(part 1 of 2)
# Autodesk Inventor assembly: testframe
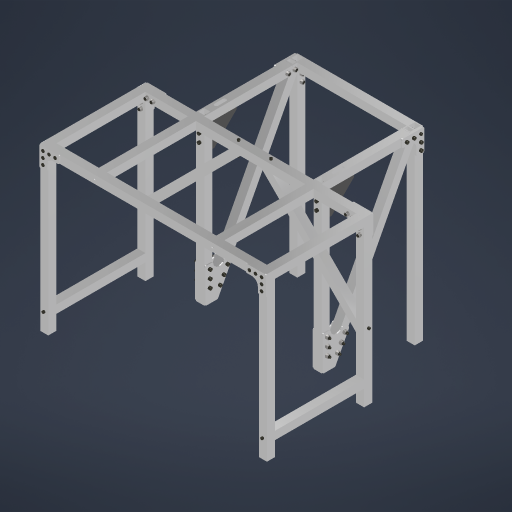
[picture p0: Inventor's stored thumbnail of the model, 512x512]
Saved by Autodesk Inventor 2024.2 (Build 282272000, 272)
## iProperties
Created: 2024-07-23
Part Number: testframe
Document SubType Name: Assembly
Designer: bryan
Mass: 9469.34 g
Surface Area: 20671.9 cm^2
Volume: 3372.68 cm^3
Density: 2.80766 g/cm^3
Author: bryan
## Documents named in this file (33)
- C:\Users\bobsb\OneDrive\Documents\GitHub\1622-2024-Summer-CAD-A-Thon\Structure\STRU_000_StructureAssembly.iam
- C:\Users\bobsb\OneDrive\Documents\GitHub\1622-2024-Summer-CAD-A-Thon\Structure\STRU_001_BilletBlock.ipt
- C:\Users\bobsb\OneDrive\Documents\GitHub\1622-2024-Summer-CAD-A-Thon\Structure\STRU_002_BilletPole_20.56in_Angled.ipt
- C:\Users\bobsb\OneDrive\Documents\GitHub\1622-2024-Summer-CAD-A-Thon\Structure\STRU_003_BilletPole_28in_Angled.ipt
- C:\Users\bobsb\OneDrive\Documents\GitHub\1622-2024-Summer-CAD-A-Thon\Structure\STRU_004_DoubleBillet_90_2.25in.ipt
- C:\Users\bobsb\OneDrive\Documents\GitHub\1622-2024-Summer-CAD-A-Thon\Structure\STRU_007_BilletPole_11in.ipt
- C:\Users\bobsb\OneDrive\Documents\GitHub\1622-2024-Summer-CAD-A-Thon\Structure\STRU_003_BilletPole_28in_Angled_Unique.ipt
- C:\Users\bobsb\OneDrive\Documents\GitHub\1622-2024-Summer-CAD-A-Thon\COTS Library\Fasteners\Bolts\Socket-Head\10-32\COTS_90044A120_Black-Oxide Alloy Steel Socket Head Screw.ipt
- C:\Users\bobsb\OneDrive\Documents\GitHub\1622-2024-Summer-CAD-A-Thon\COTS Library\Fasteners\Bolts\Socket-Head\0.25-20\COTS_90044A123_Black-Oxide Alloy Steel Socket Head Screw.ipt
- C:\Users\bobsb\OneDrive\Documents\GitHub\1622-2024-Summer-CAD-A-Thon\COTS Library\Fasteners\Nuts\COTS_95615A120_Medium-Strength Steel Nylon-Insert Locknut.ipt
- C:\Users\bobsb\OneDrive\Documents\GitHub\1622-2024-Summer-CAD-A-Thon\Structure\STRU_009_FrameBracket_90.ipt
- C:\Users\bobsb\OneDrive\Documents\GitHub\1622-2024-Summer-CAD-A-Thon\Structure\STRU_006_BilletPole_SwerveOffset.ipt
- C:\Users\bobsb\OneDrive\Documents\GitHub\1622-2024-Summer-CAD-A-Thon\Structure\STRU_010_BilletCrossbar_Angled.ipt
- C:\Users\bobsb\OneDrive\Documents\GitHub\1622-2024-Summer-CAD-A-Thon\Structure\STRU_011_BilletWedge.ipt
- C:\Users\bobsb\OneDrive\Documents\GitHub\1622-2024-Summer-CAD-A-Thon\COTS Library\Fasteners\Bolts\Socket-Head\10-32\COTS_90044A119_Black-Oxide Alloy Steel Socket Head Screw.ipt
- C:\Users\bobsb\OneDrive\Documents\GitHub\1622-2024-Summer-CAD-A-Thon\Structure\STRU_012_BilletPoleMiddle.ipt
- C:\Users\bobsb\OneDrive\Documents\GitHub\1622-2024-Summer-CAD-A-Thon\Structure\STRU_013_BilletCrossbar2_Angled.ipt
- C:\Users\bobsb\OneDrive\Documents\GitHub\1622-2024-Summer-CAD-A-Thon\Structure\STRU_012_BilletPoleMiddle_Unique.ipt
- C:\Users\bobsb\OneDrive\Documents\GitHub\1622-2024-Summer-CAD-A-Thon\Structure\STRU_014_BilletPole_9in_Angled.ipt
- C:\Users\bobsb\OneDrive\Documents\GitHub\1622-2024-Summer-CAD-A-Thon\Structure\STRU_015_BilletPole_9in.ipt
- C:\Users\bobsb\OneDrive\Documents\GitHub\1622-2024-Summer-CAD-A-Thon\Structure\STRU_016_FrameBracket2_90.ipt
- C:\Users\bobsb\OneDrive\Documents\GitHub\1622-2024-Summer-CAD-A-Thon\Structure\STRU_017_AngleBracket_90_Plastic.ipt
- C:\Users\bobsb\OneDrive\Documents\GitHub\1622-2024-Summer-CAD-A-Thon\Structure\STRU_018_AngleBracket_62.ipt
- C:\Users\bobsb\OneDrive\Documents\GitHub\1622-2024-Summer-CAD-A-Thon\COTS Library\Fasteners\Bolts\Socket-Head\0.25-20\COTS_91251A539_Black-Oxide Alloy Steel Socket Head Screw (1).ipt
- C:\Users\bobsb\OneDrive\Documents\GitHub\1622-2024-Summer-CAD-A-Thon\COTS Library\Fasteners\Bolts\Socket-Head\0.25-20\COTS_90044A124_Black-Oxide Alloy Steel Socket Head Screw.ipt
- C:\Users\bobsb\OneDrive\Documents\GitHub\1622-2024-Summer-CAD-A-Thon\COTS Library\Fasteners\Nuts\COTS_95462A029_Medium-Strength Steel Hex Nut (2).ipt
- C:\Users\bobsb\OneDrive\Documents\GitHub\1622-2024-Summer-CAD-A-Thon\Structure\STRU_019_RubberWasher.ipt
- C:\Users\bobsb\OneDrive\Documents\GitHub\1622-2024-Summer-CAD-A-Thon\Structure\STRU_023_Kenji_11in.ipt
- C:\Users\bobsb\OneDrive\Documents\GitHub\1622-2024-Summer-CAD-A-Thon\Structure\STRU_024_BilletBlock2.ipt
- C:\Users\bobsb\OneDrive\Documents\GitHub\1622-2024-Summer-CAD-A-Thon\COTS Library\Fasteners\Bolts\Socket-Head\0.25-20\COTS_90357A018_Ultra-Low-Profile Socket Head Screw.ipt
- C:\Users\bobsb\OneDrive\Documents\GitHub\1622-2024-Summer-CAD-A-Thon\COTS Library\Fasteners\Bolts\Socket-Head\0.25-20\COTS_90357A021_Ultra-Low-Profile Socket Head Screw.ipt
- C:\Users\bobsb\OneDrive\Documents\GitHub\1622-2024-Summer-CAD-A-Thon\COTS Library\Fasteners\Bolts\Socket-Head\10-32\COTS_91251A352_Black-Oxide Alloy Steel Socket Head.ipt
- C:\Users\bobsb\OneDrive\Documents\GitHub\1622-2024-Summer-CAD-A-Thon\Structure\STRU_000_StructureAssembly\AIP\FEA\err5tqxb5.fres
## Components (177 placed, 31 different names)
1. STRU_001_BilletBlock:2 — Mate:16, Mate:17, Flush:2
2. STRU_002_BilletPole_20.56in_Angled:1 — Mate:1, Mate:4, Mate:5, Mate:41, Mate:53, Mate:54, Flush:10, Mate:91, Mate:92, Mate:127, Mate:147, Mate:148, Mate:209, Mate:211, Mate:212, Mate:213, Mate:411, Mate:470, Mate:471, Flush:63, Mate:527, Mate:528
3. STRU_004_DoubleBillet_90_2.25in:1 — Mate:1, Mate:4, Mate:5, Mate:34, Mate:56, Mate:58, Mate:125, Mate:126
4. STRU_002_BilletPole_20.56in_Angled:2 — Mate:13, Mate:14, Mate:15, Mate:16, Mate:17, Flush:2, Mate:40, Mate:85, Mate:86, Mate:123, Mate:124, Mate:145, Mate:146, Mate:200, Mate:201, Mate:218, Mate:219, Mate:415, Mate:477, Mate:478, Mate:483, Mate:531, Mate:532
5. STRU_004_DoubleBillet_90_2.25in:2 — Mate:13, Mate:14, Mate:15, Mate:36, Mate:57, Mate:100, Mate:121, Mate:122
6. STRU_001_BilletBlock:3 — Mate:185, Mate:186, Flush:26
7. STRU_001_BilletBlock:4 — Mate:180, Mate:181, Flush:25
8. STRU_003_BilletPole_28in_Angled:2 — Mate:47, Flush:8, Flush:9, Mate:55, Mate:118, Mate:130, Mate:153, Mate:154, Mate:155, Mate:156, Mate:173, Flush:24, Mate:176, Mate:178, Mate:182, Mate:484, Mate:485, Mate:486, Mate:490, Flush:68, Mate:491, Mate:492, Mate:493
9. STRU_004_DoubleBillet_90_2.25in:3 — Mate:128, Mate:129, Mate:184
10. STRU_004_DoubleBillet_90_2.25in:4 — Mate:119, Mate:120, Mate:179
11. STRU_001_BilletBlock:5 — Mate:34, Mate:41, Mate:50, Mate:51, Flush:65
12. STRU_001_BilletBlock:8 — Mate:36, Mate:40, Mate:42, Mate:43
13. STRU_007_BilletPole_11in:1 — Flush:9, Mate:50, Mate:51, Mate:55, Mate:59
14. STRU_007_BilletPole_11in:2 — Mate:42, Mate:43, Mate:47, Flush:8, Mate:124
15. STRU_001_BilletBlock:9 — Mate:53, Mate:54, Flush:10
16. STRU_003_BilletPole_28in_Angled_Unique:1 — Mate:56, Mate:57, Mate:58, Mate:59, Mate:83, Mate:84, Mate:93, Mate:94, Mate:98, Mate:149, Mate:150, Mate:151, Mate:152, Mate:159, Mate:160, Mate:164, Mate:165, Flush:27, Mate:203, Mate:205, Mate:206, Mate:208, Mate:214, Mate:215, Mate:216, Mate:217, Flush:28, Mate:221, Flush:29, Mate:223, Mate:261, Mate:262, Mate:408, Mate:412, Flush:68
17. COTS_90044A123_Black-Oxide Alloy Steel Socket Head Screw:6 — Mate:84, Mate:108, Flush:12
18. COTS_90044A123_Black-Oxide Alloy Steel Socket Head Screw:7 — Mate:85, Mate:106, Mate:134, Flush:12, Flush:13, Flush:14
19. COTS_90044A123_Black-Oxide Alloy Steel Socket Head Screw:8 — Mate:83, Mate:107, Flush:13
20. COTS_90044A123_Black-Oxide Alloy Steel Socket Head Screw:9 — Mate:86, Mate:105, Flush:14
21. COTS_90044A123_Black-Oxide Alloy Steel Socket Head Screw:14 — Mate:93, Mate:115, Flush:16
22. COTS_90044A123_Black-Oxide Alloy Steel Socket Head Screw:15 — Mate:92, Mate:114, Flush:17
23. COTS_90044A123_Black-Oxide Alloy Steel Socket Head Screw:16 — Mate:91, Mate:113, Mate:136, Flush:15, Flush:17
24. COTS_90044A123_Black-Oxide Alloy Steel Socket Head Screw:17 — Mate:94, Mate:116, Flush:15, Flush:16
25. COTS_90044A120_Black-Oxide Alloy Steel Socket Head Screw:6 — Mate:100, Mate:135
26. COTS_90044A120_Black-Oxide Alloy Steel Socket Head Screw:7 — Mate:98, Mate:137
27. COTS_95615A120_Medium-Strength Steel Nylon-Insert Locknut:1 — Mate:154, Mate:522
28. COTS_95615A120_Medium-Strength Steel Nylon-Insert Locknut:2 — Mate:153, Mate:521
29. COTS_95615A120_Medium-Strength Steel Nylon-Insert Locknut:3 — Mate:194, Mate:519
30. COTS_95615A120_Medium-Strength Steel Nylon-Insert Locknut:4 — Mate:195, Mate:520
31. COTS_95615A120_Medium-Strength Steel Nylon-Insert Locknut:5 — Mate:107, Mate:152
32. COTS_95615A120_Medium-Strength Steel Nylon-Insert Locknut:6 — Mate:108, Mate:151
33. COTS_95615A120_Medium-Strength Steel Nylon-Insert Locknut:7 — Mate:105, Mate:145
34. COTS_95615A120_Medium-Strength Steel Nylon-Insert Locknut:8 — Mate:106, Mate:146
35. COTS_95615A120_Medium-Strength Steel Nylon-Insert Locknut:9 — Mate:155, Mate:514
36. COTS_95615A120_Medium-Strength Steel Nylon-Insert Locknut:10 — Mate:156, Mate:515
37. COTS_95615A120_Medium-Strength Steel Nylon-Insert Locknut:11 — Mate:189, Mate:513
38. COTS_95615A120_Medium-Strength Steel Nylon-Insert Locknut:12 — Mate:190, Mate:512
39. COTS_95615A120_Medium-Strength Steel Nylon-Insert Locknut:13 — Mate:114, Mate:147
40. COTS_95615A120_Medium-Strength Steel Nylon-Insert Locknut:14 — Mate:113, Mate:148
41. COTS_95615A120_Medium-Strength Steel Nylon-Insert Locknut:15 — Mate:115, Mate:149
42. COTS_95615A120_Medium-Strength Steel Nylon-Insert Locknut:16 — Mate:116, Mate:150
43. STRU_009_FrameBracket_90:1 — Mate:118, Mate:119, Mate:120, Mate:177, Mate:497, Mate:498, Mate:499, Mate:500, Mate:501, Mate:502, Mate:503, Mate:516, Mate:517, Mate:518
44. STRU_009_FrameBracket_90:2 — Mate:125, Mate:126, Mate:127, Mate:136, Mate:137
45. STRU_009_FrameBracket_90:3 — Mate:121, Mate:122, Mate:123, Mate:134, Mate:135
46. STRU_009_FrameBracket_90:4 — Mate:128, Mate:129, Mate:130, Mate:183, Mate:504, Mate:505, Mate:506, Mate:507, Mate:508, Mate:509, Mate:510, Mate:511, Mate:523, Mate:524
47. STRU_001_BilletBlock:11 — Mate:159, Mate:165, Mate:171
48. STRU_001_BilletBlock:12 — Mate:160, Mate:164, Mate:174, Flush:66
49. STRU_007_BilletPole_11in:3 — Mate:171, Mate:173, Flush:27
50. STRU_007_BilletPole_11in:4 — Mate:174, Flush:24, Mate:176
51. STRU_006_BilletPole_SwerveOffset:1 — Mate:177, Mate:178, Mate:179, Mate:180, Mate:181, Flush:25, Mate:194, Mate:195, Flush:64, Mate:487, Mate:489, Mate:494, Mate:529, Mate:530
52. STRU_006_BilletPole_SwerveOffset:2 — Mate:182, Mate:183, Mate:184, Mate:185, Mate:186, Flush:26, Mate:189, Mate:190, Mate:475, Mate:488, Mate:495, Mate:525, Mate:526
53. STRU_011_BilletWedge:1 — Mate:200, Mate:201, Mate:414
54. STRU_011_BilletWedge:3 — Mate:203, Mate:205, Mate:413
55. STRU_011_BilletWedge:4 — Mate:206, Mate:208, Mate:409
56. STRU_011_BilletWedge:5 — Mate:209, Mate:211, Mate:410
57. COTS_90044A119_Black-Oxide Alloy Steel Socket Head Screw:1 — Mate:212, Mate:213
58. COTS_90044A119_Black-Oxide Alloy Steel Socket Head Screw:2 — Mate:214, Mate:215
59. COTS_90044A119_Black-Oxide Alloy Steel Socket Head Screw:3 — Mate:216, Mate:217
60. COTS_90044A119_Black-Oxide Alloy Steel Socket Head Screw:4 — Mate:218, Mate:219
61. STRU_012_BilletPoleMiddle:6 — Flush:28, Mate:221, Mate:228, Mate:229, Flush:30, Flush:43, Mate:251, Mate:255, Flush:49, Mate:261, Mate:263, Mate:318, Mate:324, Mate:331, Mate:389, Mate:390, Mate:418, Mate:419
62. STRU_012_BilletPoleMiddle:5 — Flush:29, Mate:223, Mate:230, Mate:231, Flush:31, Flush:39, Mate:233, Mate:234, Mate:249, Mate:253, Flush:48, Mate:262, Mate:264, Mate:319, Mate:321, Mate:328, Mate:391, Mate:392, Mate:416, Mate:417
63. STRU_001_BilletBlock:14 — Mate:228, Mate:229, Flush:30
64. STRU_001_BilletBlock:15 — Mate:230, Mate:231, Flush:31
65. STRU_013_BilletCrossbar2_Angled:1 — Flush:39, Mate:233, Mate:234, Mate:252, Mate:273, Flush:56, Flush:57, Mate:287, Mate:322, Mate:323, Mate:327, Mate:329
66. STRU_013_BilletCrossbar2_Angled:3 — Flush:43, Mate:254, Mate:274, Flush:58, Mate:308, Mate:325, Mate:326, Mate:330, Mate:332
67. STRU_001_BilletBlock:16 — Mate:267, Mate:268, Flush:54
68. STRU_001_BilletBlock:17 — Mate:269, Mate:270, Flush:55
69. COTS_90044A120_Black-Oxide Alloy Steel Socket Head Screw:11 — Mate:249, Mate:264
70. COTS_90044A120_Black-Oxide Alloy Steel Socket Head Screw:12 — Mate:251, Mate:263
71. STRU_014_BilletPole_9in_Angled:1 — Mate:254, Mate:255, Flush:49, Mate:311, Mate:317, Mate:333, Mate:334, Mate:335, Mate:336
72. STRU_014_BilletPole_9in_Angled:2 — Mate:252, Mate:253, Flush:48, Mate:291, Mate:320, Mate:337, Mate:338, Mate:339, Mate:340
73. STRU_015_BilletPole_9in:1 — Mate:257, Mate:258, Mate:259, Mate:260, Flush:52, Flush:53, Flush:57
74. STRU_001_BilletBlock:18 — Mate:259, Mate:260, Flush:52, Mate:266, Mate:271, Mate:275
75. STRU_001_BilletBlock:19 — Mate:257, Mate:258, Flush:53, Mate:265, Mate:272, Mate:276
76. STRU_012_BilletPoleMiddle_Unique:1 — Mate:265, Mate:267, Mate:268, Flush:54, Mate:272, Mate:274, Flush:58, Mate:277, Mate:278, Mate:279, Mate:304, Mate:316
77. STRU_012_BilletPoleMiddle_Unique:2 — Mate:266, Mate:269, Mate:270, Flush:55, Mate:271, Mate:273, Flush:56, Mate:281, Mate:282, Mate:283, Mate:295, Mate:299
78. COTS_90044A120_Black-Oxide Alloy Steel Socket Head Screw:13 — Mate:275, Mate:284
79. COTS_90044A120_Black-Oxide Alloy Steel Socket Head Screw:14 — Mate:276, Mate:280
80. STRU_016_FrameBracket2_90:1 — Mate:277, Mate:278, Mate:279, Mate:280, Mate:302, Mate:303, Mate:306, Mate:307, Mate:310, Mate:312, Mate:314, Mate:315
81. STRU_016_FrameBracket2_90:2 — Mate:281, Mate:282, Mate:283, Mate:284, Mate:286, Mate:288, Mate:290, Mate:292, Mate:294, Mate:296, Mate:298, Mate:300
82. COTS_90044A123_Black-Oxide Alloy Steel Socket Head Screw:18 — Mate:286, Mate:288
83. COTS_95615A120_Medium-Strength Steel Nylon-Insert Locknut:17 — Mate:287
84. COTS_90044A123_Black-Oxide Alloy Steel Socket Head Screw:19 — Mate:290, Mate:292
85. COTS_95615A120_Medium-Strength Steel Nylon-Insert Locknut:18 — Mate:291
86. COTS_90044A123_Black-Oxide Alloy Steel Socket Head Screw:20 — Mate:294, Mate:296
87. COTS_95615A120_Medium-Strength Steel Nylon-Insert Locknut:19 — Mate:295
88. COTS_90044A123_Black-Oxide Alloy Steel Socket Head Screw:21 — Mate:298, Mate:300
89. COTS_95615A120_Medium-Strength Steel Nylon-Insert Locknut:20 — Mate:299
90. COTS_90044A123_Black-Oxide Alloy Steel Socket Head Screw:22 — Mate:302, Mate:303
91. COTS_95615A120_Medium-Strength Steel Nylon-Insert Locknut:21 — Mate:304
92. COTS_90044A123_Black-Oxide Alloy Steel Socket Head Screw:23 — Mate:306, Mate:307
93. COTS_95615A120_Medium-Strength Steel Nylon-Insert Locknut:22 — Mate:308
94. COTS_90044A123_Black-Oxide Alloy Steel Socket Head Screw:24 — Mate:310, Mate:312
95. COTS_95615A120_Medium-Strength Steel Nylon-Insert Locknut:23 — Mate:311
96. COTS_90044A123_Black-Oxide Alloy Steel Socket Head Screw:25 — Mate:314, Mate:315
97. COTS_95615A120_Medium-Strength Steel Nylon-Insert Locknut:24 — Mate:316
98. STRU_017_AngleBracket_90_Plastic:1 — Mate:317, Mate:318, Mate:453, Mate:454, Mate:458, Mate:462, Mate:463, Mate:467
99. STRU_017_AngleBracket_90_Plastic:2 — Mate:319, Mate:320, Mate:434, Mate:435, Mate:440, Mate:444, Mate:445, Mate:449
100. STRU_018_AngleBracket_62:1 — Mate:327, Mate:328, Mate:329, Mate:393, Mate:394, Mate:395, Mate:396, Mate:397, Mate:398, Mate:399, Mate:400, Mate:401, Mate:402, Mate:403, Mate:404
101. STRU_018_AngleBracket_62:2 — Mate:330, Mate:331, Mate:332, Mate:359, Mate:360, Mate:361, Mate:362, Mate:363, Mate:364, Mate:383, Mate:384, Mate:385, Mate:386, Mate:387, Mate:388
102. STRU_018_AngleBracket_62:3 — Mate:321, Mate:322, Mate:323, Mate:426, Mate:427, Mate:428, Mate:429, Mate:430, Mate:431
103. STRU_018_AngleBracket_62:4 — Mate:324, Mate:325, Mate:326, Mate:377, Mate:378, Mate:379, Mate:380, Mate:381, Mate:382
104. COTS_91251A539_Black-Oxide Alloy Steel Socket Head Screw (1):1 — Mate:337, Mate:340, Mate:439
105. COTS_91251A539_Black-Oxide Alloy Steel Socket Head Screw (1):2 — Mate:338, Mate:339, Mate:432, Mate:433
106. COTS_91251A539_Black-Oxide Alloy Steel Socket Head Screw (1):4 — Mate:333, Mate:334, Mate:457
107. COTS_91251A539_Black-Oxide Alloy Steel Socket Head Screw (1):5 — Mate:335, Mate:336, Mate:452
108. COTS_95615A120_Medium-Strength Steel Nylon-Insert Locknut:25 — Mate:373, Mate:385
109. COTS_95615A120_Medium-Strength Steel Nylon-Insert Locknut:26 — Mate:372, Mate:384
110. COTS_95615A120_Medium-Strength Steel Nylon-Insert Locknut:27 — Mate:371, Mate:383
111. COTS_95615A120_Medium-Strength Steel Nylon-Insert Locknut:28 — Mate:376, Mate:388
112. COTS_95615A120_Medium-Strength Steel Nylon-Insert Locknut:29 — Mate:375, Mate:387
113. COTS_95615A120_Medium-Strength Steel Nylon-Insert Locknut:30 — Mate:374, Mate:386
114. COTS_90044A123_Black-Oxide Alloy Steel Socket Head Screw:27 — Mate:390, Mate:419, Mate:461
115. COTS_90044A123_Black-Oxide Alloy Steel Socket Head Screw:28 — Mate:389, Mate:418, Mate:466
116. COTS_90044A123_Black-Oxide Alloy Steel Socket Head Screw:29 — Mate:392, Mate:417, Mate:448
117. COTS_90044A123_Black-Oxide Alloy Steel Socket Head Screw:30 — Mate:391, Mate:416, Mate:442, Mate:443
118. COTS_90044A124_Black-Oxide Alloy Steel Socket Head Screw:1 — Mate:359, Mate:371, Mate:382
119. COTS_90044A124_Black-Oxide Alloy Steel Socket Head Screw:2 — Mate:361, Mate:373, Mate:378
120. COTS_90044A124_Black-Oxide Alloy Steel Socket Head Screw:3 — Mate:360, Mate:372, Mate:381
121. COTS_90044A124_Black-Oxide Alloy Steel Socket Head Screw:4 — Mate:393, Mate:399, Mate:421
122. COTS_90044A124_Black-Oxide Alloy Steel Socket Head Screw:5 — Mate:394, Mate:401, Mate:422
123. COTS_90044A124_Black-Oxide Alloy Steel Socket Head Screw:6 — Mate:395, Mate:400, Mate:423
124. COTS_90044A124_Black-Oxide Alloy Steel Socket Head Screw:7 — Mate:362, Mate:374, Mate:379
125. COTS_90044A124_Black-Oxide Alloy Steel Socket Head Screw:8 — Mate:363, Mate:375, Mate:380
126. COTS_90044A124_Black-Oxide Alloy Steel Socket Head Screw:9 — Mate:364, Mate:376, Mate:377
127. COTS_90044A124_Black-Oxide Alloy Steel Socket Head Screw:10 — Mate:396, Mate:404, Mate:425
128. COTS_90044A124_Black-Oxide Alloy Steel Socket Head Screw:11 — Mate:397, Mate:403, Mate:424
129. COTS_90044A124_Black-Oxide Alloy Steel Socket Head Screw:12 — Mate:398, Mate:402, Mate:420
130. STRU_010_BilletCrossbar_Angled:2 — Mate:408, Mate:409, Mate:410, Mate:411
131. STRU_010_BilletCrossbar_Angled:3 — Mate:412, Mate:413, Mate:414, Mate:415
132. COTS_95615A120_Medium-Strength Steel Nylon-Insert Locknut:31 — Mate:423, Mate:430
133. COTS_95615A120_Medium-Strength Steel Nylon-Insert Locknut:32 — Mate:421, Mate:426
134. COTS_95615A120_Medium-Strength Steel Nylon-Insert Locknut:33 — Mate:425, Mate:429
135. COTS_95615A120_Medium-Strength Steel Nylon-Insert Locknut:34 — Mate:420, Mate:427
136. COTS_95615A120_Medium-Strength Steel Nylon-Insert Locknut:35 — Mate:422, Mate:431
137. COTS_95615A120_Medium-Strength Steel Nylon-Insert Locknut:36 — Mate:424, Mate:428
138. COTS_95462A029_Medium-Strength Steel Hex Nut (2):1 — Mate:432, Mate:436
139. STRU_019_RubberWasher:1 — Mate:433, Mate:434, Mate:435, Mate:436, Flush:59
140. COTS_95462A029_Medium-Strength Steel Hex Nut (2):2 — Mate:438, Mate:439
141. STRU_019_RubberWasher:2 — Mate:438, Flush:59, Mate:440
142. COTS_95462A029_Medium-Strength Steel Hex Nut (2):3 — Mate:442
143. STRU_019_RubberWasher:3 — Mate:443, Mate:444, Mate:445, Flush:60
144. COTS_95462A029_Medium-Strength Steel Hex Nut (2):4 — Mate:447, Mate:448
145. STRU_019_RubberWasher:4 — Mate:447, Mate:449, Flush:60
146. COTS_95462A029_Medium-Strength Steel Hex Nut (2):5 — Mate:452
147. STRU_019_RubberWasher:5 — Mate:453, Mate:454, Flush:61
148. COTS_95462A029_Medium-Strength Steel Hex Nut (2):6 — Mate:457
149. STRU_019_RubberWasher:6 — Mate:458, Flush:61
150. COTS_95462A029_Medium-Strength Steel Hex Nut (2):7 — Mate:461
151. STRU_019_RubberWasher:7 — Mate:462, Mate:463, Flush:62
152. COTS_95462A029_Medium-Strength Steel Hex Nut (2):8 — Mate:466
153. STRU_019_RubberWasher:8 — Mate:467, Flush:62
154. STRU_023_Kenji_11in:1 — Mate:472, Mate:473, Flush:63, Mate:475
155. STRU_023_Kenji_11in:2 — Flush:64, Mate:482, Mate:483, Mate:496
156. STRU_001_BilletBlock:22 — Mate:470, Mate:471, Mate:472, Mate:473
157. STRU_001_BilletBlock:23 — Mate:477, Mate:478, Mate:482
158. STRU_024_BilletBlock2:1 — Mate:484, Mate:490, Flush:65
159. STRU_024_BilletBlock2:2 — Mate:487, Flush:69, Mate:492
160. STRU_024_BilletBlock2:3 — Mate:488, Mate:495, Flush:70
161. STRU_024_BilletBlock2:4 — Mate:489, Mate:494, Flush:70, Mate:496
162. STRU_024_BilletBlock2:5 — Mate:486, Flush:67, Flush:69, Mate:491
163. STRU_024_BilletBlock2:6 — Mate:485, Flush:66, Flush:67, Mate:493
164. COTS_90357A018_Ultra-Low-Profile Socket Head Screw:1 — Mate:499, Mate:500, Mate:521
165. COTS_90357A021_Ultra-Low-Profile Socket Head Screw:1 — Mate:497, Mate:498
166. COTS_90357A018_Ultra-Low-Profile Socket Head Screw:2 — Mate:501, Mate:516, Mate:522
167. COTS_90357A018_Ultra-Low-Profile Socket Head Screw:3 — Mate:502, Mate:518, Mate:519
168. COTS_90357A018_Ultra-Low-Profile Socket Head Screw:4 — Mate:503, Mate:517, Mate:520
169. COTS_90357A018_Ultra-Low-Profile Socket Head Screw:5 — Mate:504, Mate:508, Mate:514
170. COTS_90357A018_Ultra-Low-Profile Socket Head Screw:6 — Mate:505, Mate:509, Mate:515
171. COTS_90357A018_Ultra-Low-Profile Socket Head Screw:7 — Mate:506, Mate:510, Mate:513
172. COTS_90357A018_Ultra-Low-Profile Socket Head Screw:8 — Mate:507, Mate:511, Mate:512
173. COTS_90357A021_Ultra-Low-Profile Socket Head Screw:2 — Mate:523, Mate:524
174. COTS_91251A352_Black-Oxide Alloy Steel Socket Head:1 — Mate:525, Mate:526
175. COTS_91251A352_Black-Oxide Alloy Steel Socket Head:2 — Mate:527, Mate:528
176. COTS_91251A352_Black-Oxide Alloy Steel Socket Head:3 — Mate:529, Mate:530
177. COTS_91251A352_Black-Oxide Alloy Steel Socket Head:4 — Mate:531, Mate:532
## Relationships (412: Mate 371, Flush 41)
- Mate:1: STRU_002_BilletPole_20.56in_Angled:1 ↔ STRU_004_DoubleBillet_90_2.25in:1
- Mate:4: STRU_002_BilletPole_20.56in_Angled:1 ↔ STRU_004_DoubleBillet_90_2.25in:1
- Mate:5: STRU_002_BilletPole_20.56in_Angled:1 ↔ STRU_004_DoubleBillet_90_2.25in:1
- Mate:13: STRU_002_BilletPole_20.56in_Angled:2 ↔ STRU_004_DoubleBillet_90_2.25in:2
- Mate:14: STRU_002_BilletPole_20.56in_Angled:2 ↔ STRU_004_DoubleBillet_90_2.25in:2
- Mate:15: STRU_002_BilletPole_20.56in_Angled:2 ↔ STRU_004_DoubleBillet_90_2.25in:2
- Mate:16: STRU_001_BilletBlock:2 ↔ STRU_002_BilletPole_20.56in_Angled:2
- Mate:17: STRU_001_BilletBlock:2 ↔ STRU_002_BilletPole_20.56in_Angled:2
- Flush:2: STRU_001_BilletBlock:2 ↔ STRU_002_BilletPole_20.56in_Angled:2
- [Mate]: STRU_003_BilletPole_28in_Angled:2 ↔ STRU_004_DoubleBillet_90_2.25in:3
- [Mate]: STRU_003_BilletPole_28in_Angled:2 ↔ STRU_004_DoubleBillet_90_2.25in:3
- [Mate]: STRU_003_BilletPole_28in_Angled:2 ↔ STRU_004_DoubleBillet_90_2.25in:3
- [Mate]: STRU_003_BilletPole_28in_Angled:2 ↔ STRU_004_DoubleBillet_90_2.25in:4
- [Mate]: STRU_003_BilletPole_28in_Angled:2 ↔ STRU_004_DoubleBillet_90_2.25in:4
- [Mate]: STRU_003_BilletPole_28in_Angled:2 ↔ STRU_004_DoubleBillet_90_2.25in:4
- Mate:34: STRU_004_DoubleBillet_90_2.25in:1 ↔ STRU_001_BilletBlock:5
- Mate:36: STRU_004_DoubleBillet_90_2.25in:2 ↔ STRU_001_BilletBlock:8
- Mate:40: STRU_002_BilletPole_20.56in_Angled:2 ↔ STRU_001_BilletBlock:8
- Mate:41: STRU_002_BilletPole_20.56in_Angled:1 ↔ STRU_001_BilletBlock:5
- Mate:42: STRU_001_BilletBlock:8 ↔ STRU_007_BilletPole_11in:2
- Mate:43: STRU_001_BilletBlock:8 ↔ STRU_007_BilletPole_11in:2
- Mate:47: STRU_003_BilletPole_28in_Angled:2 ↔ STRU_007_BilletPole_11in:2
- Flush:8: STRU_003_BilletPole_28in_Angled:2 ↔ STRU_007_BilletPole_11in:2
- Flush:9: STRU_003_BilletPole_28in_Angled:2 ↔ STRU_007_BilletPole_11in:1
- Mate:50: STRU_001_BilletBlock:5 ↔ STRU_007_BilletPole_11in:1
- Mate:51: STRU_001_BilletBlock:5 ↔ STRU_007_BilletPole_11in:1
- Mate:53: STRU_002_BilletPole_20.56in_Angled:1 ↔ STRU_001_BilletBlock:9
- Mate:54: STRU_002_BilletPole_20.56in_Angled:1 ↔ STRU_001_BilletBlock:9
- Flush:10: STRU_002_BilletPole_20.56in_Angled:1 ↔ STRU_001_BilletBlock:9
- Mate:55: STRU_003_BilletPole_28in_Angled:2 ↔ STRU_007_BilletPole_11in:1
- Mate:56: STRU_004_DoubleBillet_90_2.25in:1 ↔ STRU_003_BilletPole_28in_Angled_Unique:1
- Mate:57: STRU_004_DoubleBillet_90_2.25in:2 ↔ STRU_003_BilletPole_28in_Angled_Unique:1
- Mate:58: STRU_004_DoubleBillet_90_2.25in:1 ↔ STRU_003_BilletPole_28in_Angled_Unique:1
- Mate:59: STRU_007_BilletPole_11in:1 ↔ STRU_003_BilletPole_28in_Angled_Unique:1
- Mate:83: STRU_003_BilletPole_28in_Angled_Unique:1 ↔ COTS_90044A123_Black-Oxide Alloy Steel Socket Head Screw:8
- Mate:84: STRU_003_BilletPole_28in_Angled_Unique:1 ↔ COTS_90044A123_Black-Oxide Alloy Steel Socket Head Screw:6
- Mate:85: STRU_002_BilletPole_20.56in_Angled:2 ↔ COTS_90044A123_Black-Oxide Alloy Steel Socket Head Screw:7
- Mate:86: STRU_002_BilletPole_20.56in_Angled:2 ↔ COTS_90044A123_Black-Oxide Alloy Steel Socket Head Screw:9
- Mate:91: STRU_002_BilletPole_20.56in_Angled:1 ↔ COTS_90044A123_Black-Oxide Alloy Steel Socket Head Screw:16
- Mate:92: STRU_002_BilletPole_20.56in_Angled:1 ↔ COTS_90044A123_Black-Oxide Alloy Steel Socket Head Screw:15
- Mate:93: STRU_003_BilletPole_28in_Angled_Unique:1 ↔ COTS_90044A123_Black-Oxide Alloy Steel Socket Head Screw:14
- Mate:94: STRU_003_BilletPole_28in_Angled_Unique:1 ↔ COTS_90044A123_Black-Oxide Alloy Steel Socket Head Screw:17
- Mate:98: STRU_003_BilletPole_28in_Angled_Unique:1 ↔ COTS_90044A120_Black-Oxide Alloy Steel Socket Head Screw:7
- Mate:100: STRU_004_DoubleBillet_90_2.25in:2 ↔ COTS_90044A120_Black-Oxide Alloy Steel Socket Head Screw:6
- Mate:105: COTS_90044A123_Black-Oxide Alloy Steel Socket Head Screw:9 ↔ COTS_95615A120_Medium-Strength Steel Nylon-Insert Locknut:7
- Mate:106: COTS_90044A123_Black-Oxide Alloy Steel Socket Head Screw:7 ↔ COTS_95615A120_Medium-Strength Steel Nylon-Insert Locknut:8
- Mate:107: COTS_90044A123_Black-Oxide Alloy Steel Socket Head Screw:8 ↔ COTS_95615A120_Medium-Strength Steel Nylon-Insert Locknut:5
- Mate:108: COTS_90044A123_Black-Oxide Alloy Steel Socket Head Screw:6 ↔ COTS_95615A120_Medium-Strength Steel Nylon-Insert Locknut:6
- Mate:113: COTS_90044A123_Black-Oxide Alloy Steel Socket Head Screw:16 ↔ COTS_95615A120_Medium-Strength Steel Nylon-Insert Locknut:14
- Mate:114: COTS_90044A123_Black-Oxide Alloy Steel Socket Head Screw:15 ↔ COTS_95615A120_Medium-Strength Steel Nylon-Insert Locknut:13
- Mate:115: COTS_90044A123_Black-Oxide Alloy Steel Socket Head Screw:14 ↔ COTS_95615A120_Medium-Strength Steel Nylon-Insert Locknut:15
- Mate:116: COTS_90044A123_Black-Oxide Alloy Steel Socket Head Screw:17 ↔ COTS_95615A120_Medium-Strength Steel Nylon-Insert Locknut:16
- Mate:118: STRU_003_BilletPole_28in_Angled:2 ↔ STRU_009_FrameBracket_90:1
- Mate:119: STRU_004_DoubleBillet_90_2.25in:4 ↔ STRU_009_FrameBracket_90:1
- Mate:120: STRU_004_DoubleBillet_90_2.25in:4 ↔ STRU_009_FrameBracket_90:1
- Mate:121: STRU_004_DoubleBillet_90_2.25in:2 ↔ STRU_009_FrameBracket_90:3
- Mate:122: STRU_004_DoubleBillet_90_2.25in:2 ↔ STRU_009_FrameBracket_90:3
- Mate:123: STRU_002_BilletPole_20.56in_Angled:2 ↔ STRU_009_FrameBracket_90:3
- Mate:124: STRU_002_BilletPole_20.56in_Angled:2 ↔ STRU_007_BilletPole_11in:2
- Mate:125: STRU_004_DoubleBillet_90_2.25in:1 ↔ STRU_009_FrameBracket_90:2
- Mate:126: STRU_004_DoubleBillet_90_2.25in:1 ↔ STRU_009_FrameBracket_90:2
- Mate:127: STRU_002_BilletPole_20.56in_Angled:1 ↔ STRU_009_FrameBracket_90:2
- Mate:128: STRU_004_DoubleBillet_90_2.25in:3 ↔ STRU_009_FrameBracket_90:4
- Mate:129: STRU_004_DoubleBillet_90_2.25in:3 ↔ STRU_009_FrameBracket_90:4
- Mate:130: STRU_003_BilletPole_28in_Angled:2 ↔ STRU_009_FrameBracket_90:4
- Mate:134: COTS_90044A123_Black-Oxide Alloy Steel Socket Head Screw:7 ↔ STRU_009_FrameBracket_90:3
- Flush:12: COTS_90044A123_Black-Oxide Alloy Steel Socket Head Screw:6 ↔ COTS_90044A123_Black-Oxide Alloy Steel Socket Head Screw:7
- Mate:135: COTS_90044A120_Black-Oxide Alloy Steel Socket Head Screw:6 ↔ STRU_009_FrameBracket_90:3
- Flush:13: COTS_90044A123_Black-Oxide Alloy Steel Socket Head Screw:7 ↔ COTS_90044A123_Black-Oxide Alloy Steel Socket Head Screw:8
- Flush:14: COTS_90044A123_Black-Oxide Alloy Steel Socket Head Screw:7 ↔ COTS_90044A123_Black-Oxide Alloy Steel Socket Head Screw:9
- Mate:136: COTS_90044A123_Black-Oxide Alloy Steel Socket Head Screw:16 ↔ STRU_009_FrameBracket_90:2
- Mate:137: COTS_90044A120_Black-Oxide Alloy Steel Socket Head Screw:7 ↔ STRU_009_FrameBracket_90:2
- Flush:15: COTS_90044A123_Black-Oxide Alloy Steel Socket Head Screw:16 ↔ COTS_90044A123_Black-Oxide Alloy Steel Socket Head Screw:17
- Flush:16: COTS_90044A123_Black-Oxide Alloy Steel Socket Head Screw:14 ↔ COTS_90044A123_Black-Oxide Alloy Steel Socket Head Screw:17
- Flush:17: COTS_90044A123_Black-Oxide Alloy Steel Socket Head Screw:15 ↔ COTS_90044A123_Black-Oxide Alloy Steel Socket Head Screw:16
- Mate:145: STRU_002_BilletPole_20.56in_Angled:2 ↔ COTS_95615A120_Medium-Strength Steel Nylon-Insert Locknut:7
- Mate:146: STRU_002_BilletPole_20.56in_Angled:2 ↔ COTS_95615A120_Medium-Strength Steel Nylon-Insert Locknut:8
- Mate:147: STRU_002_BilletPole_20.56in_Angled:1 ↔ COTS_95615A120_Medium-Strength Steel Nylon-Insert Locknut:13
- Mate:148: STRU_002_BilletPole_20.56in_Angled:1 ↔ COTS_95615A120_Medium-Strength Steel Nylon-Insert Locknut:14
- Mate:149: STRU_003_BilletPole_28in_Angled_Unique:1 ↔ COTS_95615A120_Medium-Strength Steel Nylon-Insert Locknut:15
- Mate:150: STRU_003_BilletPole_28in_Angled_Unique:1 ↔ COTS_95615A120_Medium-Strength Steel Nylon-Insert Locknut:16
- Mate:151: STRU_003_BilletPole_28in_Angled_Unique:1 ↔ COTS_95615A120_Medium-Strength Steel Nylon-Insert Locknut:6
- Mate:152: STRU_003_BilletPole_28in_Angled_Unique:1 ↔ COTS_95615A120_Medium-Strength Steel Nylon-Insert Locknut:5
- Mate:153: STRU_003_BilletPole_28in_Angled:2 ↔ COTS_95615A120_Medium-Strength Steel Nylon-Insert Locknut:2
- Mate:154: STRU_003_BilletPole_28in_Angled:2 ↔ COTS_95615A120_Medium-Strength Steel Nylon-Insert Locknut:1
- Mate:155: STRU_003_BilletPole_28in_Angled:2 ↔ COTS_95615A120_Medium-Strength Steel Nylon-Insert Locknut:9
- Mate:156: STRU_003_BilletPole_28in_Angled:2 ↔ COTS_95615A120_Medium-Strength Steel Nylon-Insert Locknut:10
- Mate:159: STRU_003_BilletPole_28in_Angled_Unique:1 ↔ STRU_001_BilletBlock:11
- Mate:160: STRU_003_BilletPole_28in_Angled_Unique:1 ↔ STRU_001_BilletBlock:12
- Mate:164: STRU_003_BilletPole_28in_Angled_Unique:1 ↔ STRU_001_BilletBlock:12
- Mate:165: STRU_003_BilletPole_28in_Angled_Unique:1 ↔ STRU_001_BilletBlock:11
- Mate:171: STRU_001_BilletBlock:11 ↔ STRU_007_BilletPole_11in:3
- Mate:173: STRU_003_BilletPole_28in_Angled:2 ↔ STRU_007_BilletPole_11in:3
- Mate:174: STRU_001_BilletBlock:12 ↔ STRU_007_BilletPole_11in:4
- Flush:24: STRU_003_BilletPole_28in_Angled:2 ↔ STRU_007_BilletPole_11in:4
- Mate:176: STRU_003_BilletPole_28in_Angled:2 ↔ STRU_007_BilletPole_11in:4
- Mate:177: STRU_009_FrameBracket_90:1 ↔ STRU_006_BilletPole_SwerveOffset:1
- Mate:178: STRU_003_BilletPole_28in_Angled:2 ↔ STRU_006_BilletPole_SwerveOffset:1
- Mate:179: STRU_004_DoubleBillet_90_2.25in:4 ↔ STRU_006_BilletPole_SwerveOffset:1
- Mate:180: STRU_001_BilletBlock:4 ↔ STRU_006_BilletPole_SwerveOffset:1
- Mate:181: STRU_001_BilletBlock:4 ↔ STRU_006_BilletPole_SwerveOffset:1
- Flush:25: STRU_001_BilletBlock:4 ↔ STRU_006_BilletPole_SwerveOffset:1
- Mate:182: STRU_003_BilletPole_28in_Angled:2 ↔ STRU_006_BilletPole_SwerveOffset:2
- Mate:183: STRU_009_FrameBracket_90:4 ↔ STRU_006_BilletPole_SwerveOffset:2
- Mate:184: STRU_004_DoubleBillet_90_2.25in:3 ↔ STRU_006_BilletPole_SwerveOffset:2
- Mate:185: STRU_001_BilletBlock:3 ↔ STRU_006_BilletPole_SwerveOffset:2
- Mate:186: STRU_001_BilletBlock:3 ↔ STRU_006_BilletPole_SwerveOffset:2
- Flush:26: STRU_001_BilletBlock:3 ↔ STRU_006_BilletPole_SwerveOffset:2
- Mate:189: COTS_95615A120_Medium-Strength Steel Nylon-Insert Locknut:11 ↔ STRU_006_BilletPole_SwerveOffset:2
- Mate:190: COTS_95615A120_Medium-Strength Steel Nylon-Insert Locknut:12 ↔ STRU_006_BilletPole_SwerveOffset:2
- Mate:194: COTS_95615A120_Medium-Strength Steel Nylon-Insert Locknut:3 ↔ STRU_006_BilletPole_SwerveOffset:1
- Mate:195: COTS_95615A120_Medium-Strength Steel Nylon-Insert Locknut:4 ↔ STRU_006_BilletPole_SwerveOffset:1
- Flush:27: STRU_003_BilletPole_28in_Angled_Unique:1 ↔ STRU_007_BilletPole_11in:3
- Mate:200: STRU_002_BilletPole_20.56in_Angled:2 ↔ STRU_011_BilletWedge:1
- Mate:201: STRU_002_BilletPole_20.56in_Angled:2 ↔ STRU_011_BilletWedge:1
- Mate:203: STRU_003_BilletPole_28in_Angled_Unique:1 ↔ STRU_011_BilletWedge:3
- Mate:205: STRU_003_BilletPole_28in_Angled_Unique:1 ↔ STRU_011_BilletWedge:3
- Mate:206: STRU_003_BilletPole_28in_Angled_Unique:1 ↔ STRU_011_BilletWedge:4
- Mate:208: STRU_003_BilletPole_28in_Angled_Unique:1 ↔ STRU_011_BilletWedge:4
- Mate:209: STRU_002_BilletPole_20.56in_Angled:1 ↔ STRU_011_BilletWedge:5
- Mate:211: STRU_002_BilletPole_20.56in_Angled:1 ↔ STRU_011_BilletWedge:5
- Mate:212: STRU_002_BilletPole_20.56in_Angled:1 ↔ COTS_90044A119_Black-Oxide Alloy Steel Socket Head Screw:1
- Mate:213: STRU_002_BilletPole_20.56in_Angled:1 ↔ COTS_90044A119_Black-Oxide Alloy Steel Socket Head Screw:1
- Mate:214: STRU_003_BilletPole_28in_Angled_Unique:1 ↔ COTS_90044A119_Black-Oxide Alloy Steel Socket Head Screw:2
- Mate:215: STRU_003_BilletPole_28in_Angled_Unique:1 ↔ COTS_90044A119_Black-Oxide Alloy Steel Socket Head Screw:2
- Mate:216: STRU_003_BilletPole_28in_Angled_Unique:1 ↔ COTS_90044A119_Black-Oxide Alloy Steel Socket Head Screw:3
- Mate:217: STRU_003_BilletPole_28in_Angled_Unique:1 ↔ COTS_90044A119_Black-Oxide Alloy Steel Socket Head Screw:3
- Mate:218: STRU_002_BilletPole_20.56in_Angled:2 ↔ COTS_90044A119_Black-Oxide Alloy Steel Socket Head Screw:4
- Mate:219: STRU_002_BilletPole_20.56in_Angled:2 ↔ COTS_90044A119_Black-Oxide Alloy Steel Socket Head Screw:4
- Flush:28: STRU_003_BilletPole_28in_Angled_Unique:1 ↔ STRU_012_BilletPoleMiddle:6
- Mate:221: STRU_003_BilletPole_28in_Angled_Unique:1 ↔ STRU_012_BilletPoleMiddle:6
- Flush:29: STRU_003_BilletPole_28in_Angled_Unique:1 ↔ STRU_012_BilletPoleMiddle:5
- Mate:223: STRU_003_BilletPole_28in_Angled_Unique:1 ↔ STRU_012_BilletPoleMiddle:5
- Mate:228: STRU_012_BilletPoleMiddle:6 ↔ STRU_001_BilletBlock:14
- Mate:229: STRU_012_BilletPoleMiddle:6 ↔ STRU_001_BilletBlock:14
- Flush:30: STRU_012_BilletPoleMiddle:6 ↔ STRU_001_BilletBlock:14
- Mate:230: STRU_012_BilletPoleMiddle:5 ↔ STRU_001_BilletBlock:15
- Mate:231: STRU_012_BilletPoleMiddle:5 ↔ STRU_001_BilletBlock:15
- Flush:31: STRU_012_BilletPoleMiddle:5 ↔ STRU_001_BilletBlock:15
- Flush:39: STRU_012_BilletPoleMiddle:5 ↔ STRU_013_BilletCrossbar2_Angled:1
- Mate:233: STRU_012_BilletPoleMiddle:5 ↔ STRU_013_BilletCrossbar2_Angled:1
- Mate:234: STRU_012_BilletPoleMiddle:5 ↔ STRU_013_BilletCrossbar2_Angled:1
- Flush:43: STRU_012_BilletPoleMiddle:6 ↔ STRU_013_BilletCrossbar2_Angled:3
- Mate:249: STRU_012_BilletPoleMiddle:5 ↔ COTS_90044A120_Black-Oxide Alloy Steel Socket Head Screw:11
- Mate:251: STRU_012_BilletPoleMiddle:6 ↔ COTS_90044A120_Black-Oxide Alloy Steel Socket Head Screw:12
- Mate:252: STRU_013_BilletCrossbar2_Angled:1 ↔ STRU_014_BilletPole_9in_Angled:2
- Mate:253: STRU_012_BilletPoleMiddle:5 ↔ STRU_014_BilletPole_9in_Angled:2
- Flush:48: STRU_012_BilletPoleMiddle:5 ↔ STRU_014_BilletPole_9in_Angled:2
- Mate:254: STRU_013_BilletCrossbar2_Angled:3 ↔ STRU_014_BilletPole_9in_Angled:1
- Mate:255: STRU_012_BilletPoleMiddle:6 ↔ STRU_014_BilletPole_9in_Angled:1
- Flush:49: STRU_012_BilletPoleMiddle:6 ↔ STRU_014_BilletPole_9in_Angled:1
- Mate:257: STRU_015_BilletPole_9in:1 ↔ STRU_001_BilletBlock:19
- Mate:258: STRU_015_BilletPole_9in:1 ↔ STRU_001_BilletBlock:19
- Mate:259: STRU_015_BilletPole_9in:1 ↔ STRU_001_BilletBlock:18
- Mate:260: STRU_015_BilletPole_9in:1 ↔ STRU_001_BilletBlock:18
- Flush:52: STRU_015_BilletPole_9in:1 ↔ STRU_001_BilletBlock:18
- Flush:53: STRU_015_BilletPole_9in:1 ↔ STRU_001_BilletBlock:19
- Mate:261: STRU_003_BilletPole_28in_Angled_Unique:1 ↔ STRU_012_BilletPoleMiddle:6
- Mate:262: STRU_003_BilletPole_28in_Angled_Unique:1 ↔ STRU_012_BilletPoleMiddle:5
- Mate:263: STRU_012_BilletPoleMiddle:6 ↔ COTS_90044A120_Black-Oxide Alloy Steel Socket Head Screw:12
- Mate:264: STRU_012_BilletPoleMiddle:5 ↔ COTS_90044A120_Black-Oxide Alloy Steel Socket Head Screw:11
- Mate:265: STRU_001_BilletBlock:19 ↔ STRU_012_BilletPoleMiddle_Unique:1
- Mate:266: STRU_001_BilletBlock:18 ↔ STRU_012_BilletPoleMiddle_Unique:2
- Mate:267: STRU_001_BilletBlock:16 ↔ STRU_012_BilletPoleMiddle_Unique:1
- Mate:268: STRU_001_BilletBlock:16 ↔ STRU_012_BilletPoleMiddle_Unique:1
- Flush:54: STRU_001_BilletBlock:16 ↔ STRU_012_BilletPoleMiddle_Unique:1
- Mate:269: STRU_001_BilletBlock:17 ↔ STRU_012_BilletPoleMiddle_Unique:2
- Mate:270: STRU_001_BilletBlock:17 ↔ STRU_012_BilletPoleMiddle_Unique:2
- Flush:55: STRU_001_BilletBlock:17 ↔ STRU_012_BilletPoleMiddle_Unique:2
- Mate:271: STRU_001_BilletBlock:18 ↔ STRU_012_BilletPoleMiddle_Unique:2
- Mate:272: STRU_001_BilletBlock:19 ↔ STRU_012_BilletPoleMiddle_Unique:1
- Mate:273: STRU_013_BilletCrossbar2_Angled:1 ↔ STRU_012_BilletPoleMiddle_Unique:2
- Flush:56: STRU_013_BilletCrossbar2_Angled:1 ↔ STRU_012_BilletPoleMiddle_Unique:2
- Flush:57: STRU_013_BilletCrossbar2_Angled:1 ↔ STRU_015_BilletPole_9in:1
- Mate:274: STRU_013_BilletCrossbar2_Angled:3 ↔ STRU_012_BilletPoleMiddle_Unique:1
- Flush:58: STRU_013_BilletCrossbar2_Angled:3 ↔ STRU_012_BilletPoleMiddle_Unique:1
- Mate:275: STRU_001_BilletBlock:18 ↔ COTS_90044A120_Black-Oxide Alloy Steel Socket Head Screw:13
- Mate:276: STRU_001_BilletBlock:19 ↔ COTS_90044A120_Black-Oxide Alloy Steel Socket Head Screw:14
- Mate:277: STRU_012_BilletPoleMiddle_Unique:1 ↔ STRU_016_FrameBracket2_90:1
- Mate:278: STRU_012_BilletPoleMiddle_Unique:1 ↔ STRU_016_FrameBracket2_90:1
- Mate:279: STRU_012_BilletPoleMiddle_Unique:1 ↔ STRU_016_FrameBracket2_90:1
- Mate:280: COTS_90044A120_Black-Oxide Alloy Steel Socket Head Screw:14 ↔ STRU_016_FrameBracket2_90:1
- Mate:281: STRU_012_BilletPoleMiddle_Unique:2 ↔ STRU_016_FrameBracket2_90:2
- Mate:282: STRU_012_BilletPoleMiddle_Unique:2 ↔ STRU_016_FrameBracket2_90:2
- Mate:283: STRU_012_BilletPoleMiddle_Unique:2 ↔ STRU_016_FrameBracket2_90:2
- Mate:284: COTS_90044A120_Black-Oxide Alloy Steel Socket Head Screw:13 ↔ STRU_016_FrameBracket2_90:2
- [Mate]: COTS_90044A123_Black-Oxide Alloy Steel Socket Head Screw:18 ↔ COTS_95615A120_Medium-Strength Steel Nylon-Insert Locknut:17
- Mate:286: STRU_016_FrameBracket2_90:2 ↔ COTS_90044A123_Black-Oxide Alloy Steel Socket Head Screw:18
- Mate:287: STRU_013_BilletCrossbar2_Angled:1 ↔ COTS_95615A120_Medium-Strength Steel Nylon-Insert Locknut:17
- Mate:288: STRU_016_FrameBracket2_90:2 ↔ COTS_90044A123_Black-Oxide Alloy Steel Socket Head Screw:18
- [Mate]: COTS_90044A123_Black-Oxide Alloy Steel Socket Head Screw:19 ↔ COTS_95615A120_Medium-Strength Steel Nylon-Insert Locknut:18
- Mate:290: STRU_016_FrameBracket2_90:2 ↔ COTS_90044A123_Black-Oxide Alloy Steel Socket Head Screw:19
- Mate:291: STRU_014_BilletPole_9in_Angled:2 ↔ COTS_95615A120_Medium-Strength Steel Nylon-Insert Locknut:18
- Mate:292: STRU_016_FrameBracket2_90:2 ↔ COTS_90044A123_Black-Oxide Alloy Steel Socket Head Screw:19
- [Mate]: COTS_90044A123_Black-Oxide Alloy Steel Socket Head Screw:20 ↔ COTS_95615A120_Medium-Strength Steel Nylon-Insert Locknut:19
- Mate:294: STRU_016_FrameBracket2_90:2 ↔ COTS_90044A123_Black-Oxide Alloy Steel Socket Head Screw:20
- Mate:295: STRU_012_BilletPoleMiddle_Unique:2 ↔ COTS_95615A120_Medium-Strength Steel Nylon-Insert Locknut:19
- Mate:296: STRU_016_FrameBracket2_90:2 ↔ COTS_90044A123_Black-Oxide Alloy Steel Socket Head Screw:20
- [Mate]: COTS_90044A123_Black-Oxide Alloy Steel Socket Head Screw:21 ↔ COTS_95615A120_Medium-Strength Steel Nylon-Insert Locknut:20
- Mate:298: STRU_016_FrameBracket2_90:2 ↔ COTS_90044A123_Black-Oxide Alloy Steel Socket Head Screw:21
- Mate:299: STRU_012_BilletPoleMiddle_Unique:2 ↔ COTS_95615A120_Medium-Strength Steel Nylon-Insert Locknut:20
- Mate:300: STRU_016_FrameBracket2_90:2 ↔ COTS_90044A123_Black-Oxide Alloy Steel Socket Head Screw:21
- [Mate]: COTS_90044A123_Black-Oxide Alloy Steel Socket Head Screw:22 ↔ COTS_95615A120_Medium-Strength Steel Nylon-Insert Locknut:21
- Mate:302: STRU_016_FrameBracket2_90:1 ↔ COTS_90044A123_Black-Oxide Alloy Steel Socket Head Screw:22
- Mate:303: STRU_016_FrameBracket2_90:1 ↔ COTS_90044A123_Black-Oxide Alloy Steel Socket Head Screw:22
- Mate:304: STRU_012_BilletPoleMiddle_Unique:1 ↔ COTS_95615A120_Medium-Strength Steel Nylon-Insert Locknut:21
- [Mate]: COTS_90044A123_Black-Oxide Alloy Steel Socket Head Screw:23 ↔ COTS_95615A120_Medium-Strength Steel Nylon-Insert Locknut:22
- Mate:306: STRU_016_FrameBracket2_90:1 ↔ COTS_90044A123_Black-Oxide Alloy Steel Socket Head Screw:23
- Mate:307: STRU_016_FrameBracket2_90:1 ↔ COTS_90044A123_Black-Oxide Alloy Steel Socket Head Screw:23
- Mate:308: STRU_013_BilletCrossbar2_Angled:3 ↔ COTS_95615A120_Medium-Strength Steel Nylon-Insert Locknut:22
- [Mate]: COTS_90044A123_Black-Oxide Alloy Steel Socket Head Screw:24 ↔ COTS_95615A120_Medium-Strength Steel Nylon-Insert Locknut:23
- Mate:310: STRU_016_FrameBracket2_90:1 ↔ COTS_90044A123_Black-Oxide Alloy Steel Socket Head Screw:24
- Mate:311: STRU_014_BilletPole_9in_Angled:1 ↔ COTS_95615A120_Medium-Strength Steel Nylon-Insert Locknut:23
- Mate:312: STRU_016_FrameBracket2_90:1 ↔ COTS_90044A123_Black-Oxide Alloy Steel Socket Head Screw:24
- [Mate]: COTS_90044A123_Black-Oxide Alloy Steel Socket Head Screw:25 ↔ COTS_95615A120_Medium-Strength Steel Nylon-Insert Locknut:24
- Mate:314: STRU_016_FrameBracket2_90:1 ↔ COTS_90044A123_Black-Oxide Alloy Steel Socket Head Screw:25
- Mate:315: STRU_016_FrameBracket2_90:1 ↔ COTS_90044A123_Black-Oxide Alloy Steel Socket Head Screw:25
- Mate:316: STRU_012_BilletPoleMiddle_Unique:1 ↔ COTS_95615A120_Medium-Strength Steel Nylon-Insert Locknut:24
- Mate:317: STRU_014_BilletPole_9in_Angled:1 ↔ STRU_017_AngleBracket_90_Plastic:1
- Mate:318: STRU_012_BilletPoleMiddle:6 ↔ STRU_017_AngleBracket_90_Plastic:1
- Mate:319: STRU_012_BilletPoleMiddle:5 ↔ STRU_017_AngleBracket_90_Plastic:2
- Mate:320: STRU_014_BilletPole_9in_Angled:2 ↔ STRU_017_AngleBracket_90_Plastic:2
- Mate:321: STRU_012_BilletPoleMiddle:5 ↔ STRU_018_AngleBracket_62:3
- Mate:322: STRU_013_BilletCrossbar2_Angled:1 ↔ STRU_018_AngleBracket_62:3
- Mate:323: STRU_013_BilletCrossbar2_Angled:1 ↔ STRU_018_AngleBracket_62:3
- Mate:324: STRU_012_BilletPoleMiddle:6 ↔ STRU_018_AngleBracket_62:4
- Mate:325: STRU_013_BilletCrossbar2_Angled:3 ↔ STRU_018_AngleBracket_62:4
- Mate:326: STRU_013_BilletCrossbar2_Angled:3 ↔ STRU_018_AngleBracket_62:4
- Mate:327: STRU_013_BilletCrossbar2_Angled:1 ↔ STRU_018_AngleBracket_62:1
- Mate:328: STRU_012_BilletPoleMiddle:5 ↔ STRU_018_AngleBracket_62:1
- Mate:329: STRU_013_BilletCrossbar2_Angled:1 ↔ STRU_018_AngleBracket_62:1
- Mate:330: STRU_013_BilletCrossbar2_Angled:3 ↔ STRU_018_AngleBracket_62:2
- Mate:331: STRU_012_BilletPoleMiddle:6 ↔ STRU_018_AngleBracket_62:2
- Mate:332: STRU_013_BilletCrossbar2_Angled:3 ↔ STRU_018_AngleBracket_62:2
- Mate:333: STRU_014_BilletPole_9in_Angled:1 ↔ COTS_91251A539_Black-Oxide Alloy Steel Socket Head Screw (1):4
- Mate:334: STRU_014_BilletPole_9in_Angled:1 ↔ COTS_91251A539_Black-Oxide Alloy Steel Socket Head Screw (1):4
- Mate:335: STRU_014_BilletPole_9in_Angled:1 ↔ COTS_91251A539_Black-Oxide Alloy Steel Socket Head Screw (1):5
- Mate:336: STRU_014_BilletPole_9in_Angled:1 ↔ COTS_91251A539_Black-Oxide Alloy Steel Socket Head Screw (1):5
- Mate:337: STRU_014_BilletPole_9in_Angled:2 ↔ COTS_91251A539_Black-Oxide Alloy Steel Socket Head Screw (1):1
- Mate:338: STRU_014_BilletPole_9in_Angled:2 ↔ COTS_91251A539_Black-Oxide Alloy Steel Socket Head Screw (1):2
- Mate:339: STRU_014_BilletPole_9in_Angled:2 ↔ COTS_91251A539_Black-Oxide Alloy Steel Socket Head Screw (1):2
- Mate:340: STRU_014_BilletPole_9in_Angled:2 ↔ COTS_91251A539_Black-Oxide Alloy Steel Socket Head Screw (1):1
- Mate:359: STRU_018_AngleBracket_62:2 ↔ COTS_90044A124_Black-Oxide Alloy Steel Socket Head Screw:1
- Mate:360: STRU_018_AngleBracket_62:2 ↔ COTS_90044A124_Black-Oxide Alloy Steel Socket Head Screw:3
- Mate:361: STRU_018_AngleBracket_62:2 ↔ COTS_90044A124_Black-Oxide Alloy Steel Socket Head Screw:2
- Mate:362: STRU_018_AngleBracket_62:2 ↔ COTS_90044A124_Black-Oxide Alloy Steel Socket Head Screw:7
- Mate:363: STRU_018_AngleBracket_62:2 ↔ COTS_90044A124_Black-Oxide Alloy Steel Socket Head Screw:8
- Mate:364: STRU_018_AngleBracket_62:2 ↔ COTS_90044A124_Black-Oxide Alloy Steel Socket Head Screw:9
- Mate:371: COTS_95615A120_Medium-Strength Steel Nylon-Insert Locknut:27 ↔ COTS_90044A124_Black-Oxide Alloy Steel Socket Head Screw:1
- Mate:372: COTS_95615A120_Medium-Strength Steel Nylon-Insert Locknut:26 ↔ COTS_90044A124_Black-Oxide Alloy Steel Socket Head Screw:3
- Mate:373: COTS_95615A120_Medium-Strength Steel Nylon-Insert Locknut:25 ↔ COTS_90044A124_Black-Oxide Alloy Steel Socket Head Screw:2
- Mate:374: COTS_95615A120_Medium-Strength Steel Nylon-Insert Locknut:30 ↔ COTS_90044A124_Black-Oxide Alloy Steel Socket Head Screw:7
- Mate:375: COTS_95615A120_Medium-Strength Steel Nylon-Insert Locknut:29 ↔ COTS_90044A124_Black-Oxide Alloy Steel Socket Head Screw:8
- Mate:376: COTS_95615A120_Medium-Strength Steel Nylon-Insert Locknut:28 ↔ COTS_90044A124_Black-Oxide Alloy Steel Socket Head Screw:9
- Mate:377: STRU_018_AngleBracket_62:4 ↔ COTS_90044A124_Black-Oxide Alloy Steel Socket Head Screw:9
- Mate:378: STRU_018_AngleBracket_62:4 ↔ COTS_90044A124_Black-Oxide Alloy Steel Socket Head Screw:2
- Mate:379: STRU_018_AngleBracket_62:4 ↔ COTS_90044A124_Black-Oxide Alloy Steel Socket Head Screw:7
- Mate:380: STRU_018_AngleBracket_62:4 ↔ COTS_90044A124_Black-Oxide Alloy Steel Socket Head Screw:8
- Mate:381: STRU_018_AngleBracket_62:4 ↔ COTS_90044A124_Black-Oxide Alloy Steel Socket Head Screw:3
- Mate:382: STRU_018_AngleBracket_62:4 ↔ COTS_90044A124_Black-Oxide Alloy Steel Socket Head Screw:1
- Mate:383: STRU_018_AngleBracket_62:2 ↔ COTS_95615A120_Medium-Strength Steel Nylon-Insert Locknut:27
- Mate:384: STRU_018_AngleBracket_62:2 ↔ COTS_95615A120_Medium-Strength Steel Nylon-Insert Locknut:26
- Mate:385: STRU_018_AngleBracket_62:2 ↔ COTS_95615A120_Medium-Strength Steel Nylon-Insert Locknut:25
- Mate:386: STRU_018_AngleBracket_62:2 ↔ COTS_95615A120_Medium-Strength Steel Nylon-Insert Locknut:30
- Mate:387: STRU_018_AngleBracket_62:2 ↔ COTS_95615A120_Medium-Strength Steel Nylon-Insert Locknut:29
- Mate:388: STRU_018_AngleBracket_62:2 ↔ COTS_95615A120_Medium-Strength Steel Nylon-Insert Locknut:28
- Mate:389: STRU_012_BilletPoleMiddle:6 ↔ COTS_90044A123_Black-Oxide Alloy Steel Socket Head Screw:28
- Mate:390: STRU_012_BilletPoleMiddle:6 ↔ COTS_90044A123_Black-Oxide Alloy Steel Socket Head Screw:27
- Mate:391: STRU_012_BilletPoleMiddle:5 ↔ COTS_90044A123_Black-Oxide Alloy Steel Socket Head Screw:30
- Mate:392: STRU_012_BilletPoleMiddle:5 ↔ COTS_90044A123_Black-Oxide Alloy Steel Socket Head Screw:29
- Mate:393: STRU_018_AngleBracket_62:1 ↔ COTS_90044A124_Black-Oxide Alloy Steel Socket Head Screw:4
- Mate:394: STRU_018_AngleBracket_62:1 ↔ COTS_90044A124_Black-Oxide Alloy Steel Socket Head Screw:5
- Mate:395: STRU_018_AngleBracket_62:1 ↔ COTS_90044A124_Black-Oxide Alloy Steel Socket Head Screw:6
- Mate:396: STRU_018_AngleBracket_62:1 ↔ COTS_90044A124_Black-Oxide Alloy Steel Socket Head Screw:10
- Mate:397: STRU_018_AngleBracket_62:1 ↔ COTS_90044A124_Black-Oxide Alloy Steel Socket Head Screw:11
- Mate:398: STRU_018_AngleBracket_62:1 ↔ COTS_90044A124_Black-Oxide Alloy Steel Socket Head Screw:12
- Mate:399: STRU_018_AngleBracket_62:1 ↔ COTS_90044A124_Black-Oxide Alloy Steel Socket Head Screw:4
- Mate:400: STRU_018_AngleBracket_62:1 ↔ COTS_90044A124_Black-Oxide Alloy Steel Socket Head Screw:6
- Mate:401: STRU_018_AngleBracket_62:1 ↔ COTS_90044A124_Black-Oxide Alloy Steel Socket Head Screw:5
- Mate:402: STRU_018_AngleBracket_62:1 ↔ COTS_90044A124_Black-Oxide Alloy Steel Socket Head Screw:12
- Mate:403: STRU_018_AngleBracket_62:1 ↔ COTS_90044A124_Black-Oxide Alloy Steel Socket Head Screw:11
- Mate:404: STRU_018_AngleBracket_62:1 ↔ COTS_90044A124_Black-Oxide Alloy Steel Socket Head Screw:10
- Mate:408: STRU_003_BilletPole_28in_Angled_Unique:1 ↔ STRU_010_BilletCrossbar_Angled:2
- Mate:409: STRU_011_BilletWedge:4 ↔ STRU_010_BilletCrossbar_Angled:2
- Mate:410: STRU_011_BilletWedge:5 ↔ STRU_010_BilletCrossbar_Angled:2
- Mate:411: STRU_002_BilletPole_20.56in_Angled:1 ↔ STRU_010_BilletCrossbar_Angled:2
- Mate:412: STRU_003_BilletPole_28in_Angled_Unique:1 ↔ STRU_010_BilletCrossbar_Angled:3
- Mate:413: STRU_011_BilletWedge:3 ↔ STRU_010_BilletCrossbar_Angled:3
- Mate:414: STRU_011_BilletWedge:1 ↔ STRU_010_BilletCrossbar_Angled:3
- Mate:415: STRU_002_BilletPole_20.56in_Angled:2 ↔ STRU_010_BilletCrossbar_Angled:3
- Mate:416: STRU_012_BilletPoleMiddle:5 ↔ COTS_90044A123_Black-Oxide Alloy Steel Socket Head Screw:30
- Mate:417: STRU_012_BilletPoleMiddle:5 ↔ COTS_90044A123_Black-Oxide Alloy Steel Socket Head Screw:29
- Mate:418: STRU_012_BilletPoleMiddle:6 ↔ COTS_90044A123_Black-Oxide Alloy Steel Socket Head Screw:28
- Mate:419: STRU_012_BilletPoleMiddle:6 ↔ COTS_90044A123_Black-Oxide Alloy Steel Socket Head Screw:27
- Mate:420: COTS_90044A124_Black-Oxide Alloy Steel Socket Head Screw:12 ↔ COTS_95615A120_Medium-Strength Steel Nylon-Insert Locknut:34
- Mate:421: COTS_90044A124_Black-Oxide Alloy Steel Socket Head Screw:4 ↔ COTS_95615A120_Medium-Strength Steel Nylon-Insert Locknut:32
- Mate:422: COTS_90044A124_Black-Oxide Alloy Steel Socket Head Screw:5 ↔ COTS_95615A120_Medium-Strength Steel Nylon-Insert Locknut:35
- Mate:423: COTS_90044A124_Black-Oxide Alloy Steel Socket Head Screw:6 ↔ COTS_95615A120_Medium-Strength Steel Nylon-Insert Locknut:31
- Mate:424: COTS_90044A124_Black-Oxide Alloy Steel Socket Head Screw:11 ↔ COTS_95615A120_Medium-Strength Steel Nylon-Insert Locknut:36
- Mate:425: COTS_90044A124_Black-Oxide Alloy Steel Socket Head Screw:10 ↔ COTS_95615A120_Medium-Strength Steel Nylon-Insert Locknut:33
- Mate:426: STRU_018_AngleBracket_62:3 ↔ COTS_95615A120_Medium-Strength Steel Nylon-Insert Locknut:32